# Autodesk Inventor assembly: Assembly2
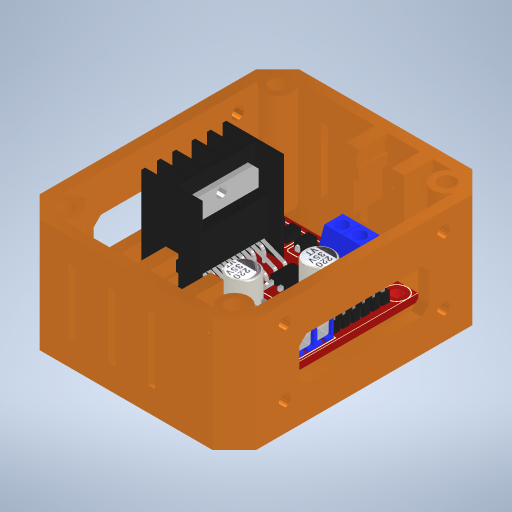
[picture p0: Inventor's stored thumbnail of the model, 512x512]
Saved by Autodesk Inventor 2024.2 (Build 282272000, 272)
## iProperties
Created: 2024-09-09
Part Number: Assembly2
Document SubType Name: Assembly
Designer: Admin
Author: Admin
## Documents named in this file (3)
- C:\Users\Admin\Documents\GitHub\ExplorateurErrant\Power\Assembly2.iam
- C:\Users\Admin\Documents\GitHub\ExplorateurErrant\Power\3DPrinted\ModuloPotencia_Cubierta.ipt
- C:\Users\Admin\Documents\GitHub\ExplorateurErrant\Power\H-Bridge\H-brug.ipt
## Components (2 placed, 2 different names)
1. ModuloPotencia_Cubierta:2 — Mate:1, Mate:2, Mate:3
2. H-brug:1 — Mate:1, Mate:2, Mate:3
## Relationships (3: Mate 3)
- Mate:1: ModuloPotencia_Cubierta:2 ↔ H-brug:1
- Mate:2: ModuloPotencia_Cubierta:2 ↔ H-brug:1
- Mate:3: ModuloPotencia_Cubierta:2 ↔ H-brug:1
